# Autodesk Inventor assembly: s-assy-guide_coupling
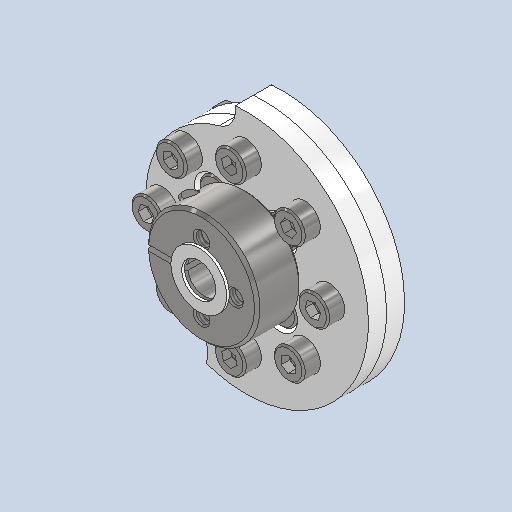
[picture p0: Inventor's stored thumbnail of the model, 512x512]
Saved by Autodesk Inventor 2022 (Build 260153000, 153)
## iProperties
Created: 2021-08-27
Part Number: s-assy-guide_coupling
Document SubType Name: Assembly
Designer: Yuta Kage
Author: Yuta Kage
## Documents named in this file (9)
- C:\Users\yuta0\Documents\GitHub\catchrobo_hardware\assy-shooter\s-assy-guide_coupling.iam
- C:\Users\yuta0\Documents\GitHub\catchrobo_hardware\assy-shooter\LBNR3.ipt
- C:\Users\yuta0\Documents\GitHub\catchrobo_hardware\assy-shooter\CB3-10.ipt
- C:\Users\yuta0\Documents\GitHub\catchrobo_hardware\assy-shooter\SCSTR6-8.iam
- C:\Users\yuta0\Documents\GitHub\catchrobo_hardware\assy-shooter\CB3-6.ipt
- C:\Users\yuta0\Documents\GitHub\catchrobo_hardware\assy-shooter\shooter_base6.ipt
- C:\Users\yuta0\Documents\GitHub\catchrobo_hardware\assy-shooter\shooter_base5.ipt
- C:\Users\yuta0\Documents\GitHub\catchrobo_hardware\assy-shooter\CC-0612-05.ipt
- C:\Users\yuta0\Documents\GitHub\catchrobo_hardware\assy-shooter\CB3-8.ipt
## Components (28 placed, 8 different names)
1. SCSTR6-8:1 [sub-assembly] — メイト:74, メイト:75, メイト:76, メイト:87, メイト:88, メイト:89
2. shooter_base6:1 — メイト:69, メイト:71, メイト:72, メイト:73, メイト:74, メイト:76, メイト:79, メイト:80, メイト:90
3. shooter_base5:1 — メイト:69, メイト:77, メイト:78, メイト:80, メイト:82, フラッシュ:1, フラッシュ:2, メイト:90
4. CC-0612-05:1 — メイト:87, メイト:88
5. CB3-6:1 — メイト:77, メイト:78
6. CB3-10:1 — メイト:72, メイト:73, メイト:75
7. CB3-6:2
8. CB3-10:3
9. CB3-6:3
10. CB3-10:4
11. CB3-6:4
12. CB3-10:5
13. CB3-8:1 — メイト:71, メイト:79, メイト:81
14. LBNR3:1 — メイト:81, メイト:82
15. CB3-8:2
16. LBNR3:2
17. CB3-8:3
18. LBNR3:3
19. CB3-8:4
20. LBNR3:4
21. CB3-8:5
22. LBNR3:5
23. CB3-8:6
24. LBNR3:6
25. CB3-8:7
26. LBNR3:7
27. CB3-8:8
28. LBNR3:8
## Component patterns: (4 elements, first: CB3-6:1 + CB3-10:1), (8 elements, first: CB3-8:1 + LBNR3:1)
## Relationships (19: Mate 17, Flush 2)
- メイト:69 [Mate]: shooter_base6:1 ↔ shooter_base5:1
- メイト:71 [Mate]: shooter_base6:1 ↔ CB3-8:1
- メイト:72 [Mate]: shooter_base6:1 ↔ CB3-10:1
- メイト:73 [Mate]: shooter_base6:1 ↔ CB3-10:1
- メイト:74 [Mate]: SCSTR6-8:1 ↔ shooter_base6:1
- メイト:75 [Mate]: SCSTR6-8:1 ↔ CB3-10:1
- メイト:76 [Mate]: SCSTR6-8:1 ↔ shooter_base6:1
- メイト:77 [Mate]: shooter_base5:1 ↔ CB3-6:1
- メイト:78 [Mate]: shooter_base5:1 ↔ CB3-6:1
- メイト:79 [Mate]: shooter_base6:1 ↔ CB3-8:1
- メイト:80 [Mate]: shooter_base6:1 ↔ shooter_base5:1
- メイト:81 [Mate]: CB3-8:1 ↔ LBNR3:1
- メイト:82 [Mate]: shooter_base5:1 ↔ LBNR3:1
- メイト:87 [Mate]: SCSTR6-8:1 ↔ CC-0612-05:1
- メイト:88 [Mate]: SCSTR6-8:1 ↔ CC-0612-05:1
- メイト:89 [Mate]: SCSTR6-8:1
- フラッシュ:1 [Flush]: shooter_base5:1
- フラッシュ:2 [Flush]: shooter_base5:1
- メイト:90 [Mate]: shooter_base6:1 ↔ shooter_base5:1
